# Autodesk Inventor assembly: Walls
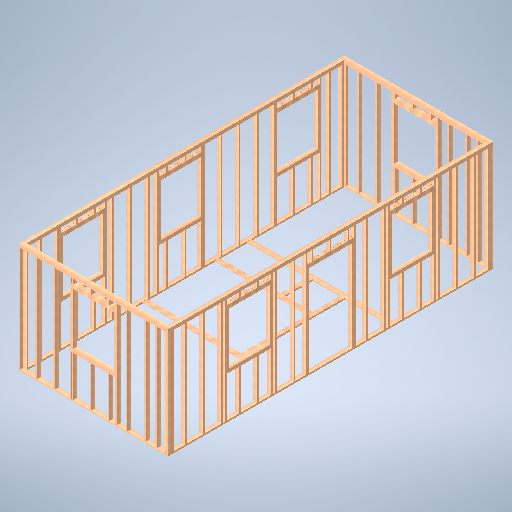
[picture p0: Inventor's stored thumbnail of the model, 512x512]
Saved by Autodesk Inventor 2025.1 (Build 291241020, 241B)
## iProperties
Created: 2024-09-15
Part Number: Walls
Document SubType Name: Assembly
Designer: Tom
Author: Tom
## Documents named in this file (19)
- C:\Users\Tom\Documents\Inventor\Mobility\Additional_Building\Framing_For_First_Floor.iam
- C:\Users\Tom\Documents\Inventor\Mobility\Additional_Building\Plate_With_Length_144_Inches.ipt
- C:\Users\Tom\Documents\Inventor\Mobility\Additional_Building\Plate_With_Length_125_Inches.ipt
- C:\Users\Tom\Documents\Inventor\Mobility\Additional_Building\California_Corner.iam
- C:\Users\Tom\Documents\Inventor\Mobility\Additional_Building\Stud_With_Height_93_Inches.ipt
- C:\Users\Tom\Documents\Inventor\Mobility\Additional_Building\Plate_With_Length_132_Inches.ipt
- C:\Users\Tom\Documents\Inventor\Mobility\Additional_Building\Plate_With_Length_68.5_Inches.ipt
- C:\Users\Tom\Documents\Inventor\Mobility\Additional_Building\Plate_With_Length_86.5625_Inches_And_Image_Of_Bath_Tub.ipt
- C:\Users\Tom\Documents\Inventor\Mobility\Additional_Building\Plate_With_Length_60_Inches.ipt
- C:\Users\Tom\Documents\Inventor\Mobility\Additional_Building\Plate_With_Length_25_Inches.ipt
- C:\Users\Tom\Documents\Inventor\Mobility\Additional_Building\Plate_With_Length_86.5625_Inches.ipt
- C:\Users\Tom\Documents\Inventor\Mobility\Additional_Building\Header_With_Dimensions_3.5_x_3.5_x_41.25_Inches.iam
- C:\Users\Tom\Documents\Inventor\Mobility\Additional_Building\Stud_With_Height_80.5_Inches.ipt
- C:\Users\Tom\Documents\Inventor\Mobility\Additional_Building\Stud_With_Height_9_Inches.ipt
- C:\Users\Tom\Documents\Inventor\Mobility\Additional_Building\Framing_For_First_Floor_Front_Window.iam
- C:\Users\Tom\Documents\Inventor\Mobility\Additional_Building\Framing_For_Side_Window.iam
- C:\Users\Tom\Documents\Inventor\Mobility\Additional_Building\Framing_For_Back_Living_Room_Window.iam
- C:\Users\Tom\Documents\Inventor\Mobility\Additional_Building\Framing_For_Bathroom_Window.iam
- C:\Users\Tom\Documents\Inventor\Mobility\Additional_Building\Framing_For_Back_Bedroom_Window.iam
## Components (74 placed, 18 different names)
1. California_Corner:1 [sub-assembly] — Mate:2, Flush:3, Flush:4
2. California_Corner:2 [sub-assembly] — Mate:13, Flush:13, Flush:14, Flush:19, Flush:20, Flush:31, Mate:34, Flush:64, Flush:70
3. California_Corner:3 [sub-assembly] — Mate:14, Flush:15, Flush:16
4. California_Corner:4 [sub-assembly] — Mate:15, Flush:17, Flush:18, Flush:74, Flush:75
5. Plate_With_Length_125_Inches:5 — Mate:16, Flush:22, Mate:17, Mate:19, Mate:24, Flush:27, Flush:45, Mate:76
6. Plate_With_Length_60_Inches:1 — Mate:19, Mate:27, Mate:31, Flush:44
7. Plate_With_Length_25_Inches:1 — Mate:25, Mate:28, Flush:45
8. Plate_With_Length_25_Inches:2 — Mate:24, Flush:27, Mate:25, Mate:29
9. Plate_With_Length_86.5625_Inches_And_Image_Of_Bath_Tub:1 — Mate:26, Flush:28, Mate:27, Mate:28, Mate:29, Flush:44
10. Plate_With_Length_86.5625_Inches:1 — Mate:30, Mate:31, Flush:29, Mate:73
11. Stud_With_Height_93_Inches:56 — Mate:33, Flush:32, Mate:34, Mate:35, Flush:33, Mate:39
12. Header_With_Dimensions_3.5_x_3.5_x_41.25_Inches:1 [sub-assembly] — Mate:35, Flush:33, Flush:34, Mate:37, Mate:42, Flush:38
13. Stud_With_Height_93_Inches:57 — Mate:36, Flush:35, Mate:37, Mate:41
14. Stud_With_Height_80.5_Inches:1 — Mate:38, Flush:36, Mate:39
15. Stud_With_Height_80.5_Inches:2 — Mate:40, Flush:37, Mate:41
16. Framing_For_First_Floor_Front_Window:1 [sub-assembly] — Mate:62, Flush:63, Flush:64
17. Framing_For_First_Floor_Front_Window:2 [sub-assembly] — Mate:63, Flush:65, Flush:66
18. Stud_With_Height_93_Inches:76 — Mate:67, Flush:73, Flush:74, Flush:79, Flush:83, Flush:85
19. Framing_For_Back_Living_Room_Window:1 [sub-assembly] — Mate:68, Flush:75, Flush:76, Mate:70
20. Stud_With_Height_93_Inches:77 — Mate:69, Flush:77, Mate:70
21. Framing_For_Bathroom_Window:1 [sub-assembly] — Mate:72, Flush:80, Mate:73
22. Framing_For_Back_Bedroom_Window:1 [sub-assembly] — Mate:74, Flush:81, Mate:76
23. Stud_With_Height_93_Inches:84 — Mate:77, Flush:84, Flush:85
24. Plate_With_Length_132_Inches:1 — Mate:8, Flush:9, Flush:10, Mate:10
25. Plate_With_Length_132_Inches:2
26. Plate_With_Length_144_Inches:9 — Mate:11, Mate:12, Flush:12
27. Plate_With_Length_144_Inches:10
28. Stud_With_Height_93_Inches:1 — Mate:4, Flush:6, Flush:19, Flush:39, Flush:43, Flush:68
29. Stud_With_Height_93_Inches:51
30. Stud_With_Height_93_Inches:60 — Flush:62
31. Stud_With_Height_9_Inches:1 — Mate:42, Flush:38, Flush:39
32. Stud_With_Height_9_Inches:2
33. Stud_With_Height_9_Inches:3
34. Stud_With_Height_93_Inches:62 — Mate:61, Flush:61, Flush:62
35. Stud_With_Height_93_Inches:63
36. Stud_With_Height_93_Inches:58 — Mate:44, Flush:42, Flush:43
37. Stud_With_Height_93_Inches:64
38. Stud_With_Height_93_Inches:65 — Mate:64, Flush:67, Flush:68
39. Stud_With_Height_93_Inches:66
40. Stud_With_Height_93_Inches:67
41. Stud_With_Height_93_Inches:49 — Mate:32, Flush:30, Flush:31
42. Framing_For_Side_Window:1 [sub-assembly] — Mate:65, Flush:69, Flush:70
43. Stud_With_Height_93_Inches:71
44. Framing_For_Side_Window:2 [sub-assembly]
45. Stud_With_Height_93_Inches:78 — Mate:71, Flush:78, Flush:79
46. Stud_With_Height_93_Inches:79
47. Stud_With_Height_93_Inches:80
48. Stud_With_Height_93_Inches:81 — Mate:75, Flush:82, Flush:83
49. Stud_With_Height_93_Inches:82
50. Stud_With_Height_93_Inches:83
51. Plate_With_Length_144_Inches:1 — Flush:5, Mate:15, Flush:17, Flush:18, Mate:30, Flush:29, Mate:67, Flush:73, Mate:68, Flush:76, Mate:69, Flush:77, Mate:71, Flush:78, Mate:72, Flush:80
52. Plate_With_Length_144_Inches:2 — Mate:14, Flush:15, Flush:16, Mate:26, Flush:28, Mate:74, Flush:81, Mate:75, Flush:82, Mate:77, Flush:84
53. Plate_With_Length_144_Inches:3 — Mate:1, Flush:1, Flush:2, Mate:4, Flush:6, Mate:13, Flush:13, Flush:14, Mate:16, Flush:22, Mate:33, Flush:32, Flush:34, Mate:38, Flush:36, Mate:61, Flush:61, Mate:62, Flush:63
54. Plate_With_Length_144_Inches:4 — Mate:2, Flush:3, Flush:4, Mate:36, Flush:35, Mate:40, Flush:37, Mate:44, Flush:42, Mate:63, Flush:65, Flush:66, Mate:64, Flush:67
55. Plate_With_Length_125_Inches:1 — Mate:1, Flush:1, Flush:2, Mate:3, Mate:7, Mate:32, Flush:30, Mate:65, Flush:69, Mate:66, Flush:71
56. Plate_With_Length_125_Inches:2 — Mate:17
57. Plate_With_Length_144_Inches:5 — Flush:9
58. Plate_With_Length_144_Inches:6
59. Plate_With_Length_144_Inches:7 — Mate:9, Flush:11
60. Plate_With_Length_144_Inches:8 — Mate:11, Flush:12
61. Plate_With_Length_125_Inches:3 — Flush:7, Mate:8, Flush:10
62. Plate_With_Length_125_Inches:4
63. Plate_With_Length_68.5_Inches:1 — Mate:9, Mate:10, Flush:11
64. Plate_With_Length_68.5_Inches:2 — Mate:12
65. Plate_With_Length_68.5_Inches:3
66. Plate_With_Length_68.5_Inches:4
67. Stud_With_Height_93_Inches:23 — Flush:7, Mate:7, Flush:20, Flush:72
68. Stud_With_Height_93_Inches:68
69. Stud_With_Height_93_Inches:69 — Mate:66, Flush:71, Flush:72
70. Stud_With_Height_93_Inches:70
71. Stud_With_Height_93_Inches:72
72. Stud_With_Height_93_Inches:73
73. Stud_With_Height_93_Inches:74
74. Stud_With_Height_93_Inches:75
## Component patterns: (2 elements), (2 elements, first: Plate_With_Length_132_Inches:1), (2 elements, first: Plate_With_Length_144_Inches:9), (3 elements, first: Stud_With_Height_93_Inches:1), (3 elements, first: Stud_With_Height_9_Inches:1), (2 elements, first: Stud_With_Height_93_Inches:62), (2 elements, first: Stud_With_Height_93_Inches:58), (3 elements, first: Stud_With_Height_93_Inches:65), (2 elements, first: Stud_With_Height_93_Inches:49 + Framing_For_Side_Window:1), (3 elements, first: Stud_With_Height_93_Inches:78), (3 elements, first: Stud_With_Height_93_Inches:81), (4 elements, first: Plate_With_Length_144_Inches:1), (2 elements, first: Plate_With_Length_125_Inches:1), Component Pattern 1:2 (4 elements), Component Pattern 2:2 (2 elements), (2 elements, first: Plate_With_Length_68.5_Inches:1), Component Pattern 10:2 (2 elements), (2 elements, first: Stud_With_Height_93_Inches:23), (2 elements, first: Stud_With_Height_93_Inches:69), Component Pattern 22:2 (2 elements), Component Pattern 23:2 (2 elements)
## Relationships (115: Flush 62, Mate 53)
- Mate:1: Plate_With_Length_144_Inches:3 ↔ Plate_With_Length_125_Inches:1
- Flush:1: Plate_With_Length_144_Inches:3 ↔ Plate_With_Length_125_Inches:1
- Flush:2: Plate_With_Length_144_Inches:3 ↔ Plate_With_Length_125_Inches:1
- Mate:2: California_Corner:1 ↔ Plate_With_Length_144_Inches:4
- Flush:3: California_Corner:1 ↔ Plate_With_Length_144_Inches:4
- Flush:4: California_Corner:1 ↔ Plate_With_Length_144_Inches:4
- Flush:5: Plate_With_Length_144_Inches:1
- Mate:3 (1536.7 mm): Plate_With_Length_125_Inches:1
- Mate:4: Stud_With_Height_93_Inches:1 ↔ Plate_With_Length_144_Inches:3
- Flush:6: Stud_With_Height_93_Inches:1 ↔ Plate_With_Length_144_Inches:3
- Flush:7: Plate_With_Length_125_Inches:3 ↔ Stud_With_Height_93_Inches:23
- Mate:7: Plate_With_Length_125_Inches:1 ↔ Stud_With_Height_93_Inches:23
- Mate:8: Plate_With_Length_132_Inches:1 ↔ Plate_With_Length_125_Inches:3
- Flush:9: Plate_With_Length_132_Inches:1 ↔ Plate_With_Length_144_Inches:5
- Flush:10: Plate_With_Length_132_Inches:1 ↔ Plate_With_Length_125_Inches:3
- Mate:9: Plate_With_Length_144_Inches:7 ↔ Plate_With_Length_68.5_Inches:1
- Mate:10: Plate_With_Length_132_Inches:1 ↔ Plate_With_Length_68.5_Inches:1
- Flush:11: Plate_With_Length_144_Inches:7 ↔ Plate_With_Length_68.5_Inches:1
- Mate:11: Plate_With_Length_144_Inches:9 ↔ Plate_With_Length_144_Inches:8
- Mate:12: Plate_With_Length_144_Inches:9 ↔ Plate_With_Length_68.5_Inches:2
- Flush:12: Plate_With_Length_144_Inches:9 ↔ Plate_With_Length_144_Inches:8
- Mate:13: California_Corner:2 ↔ Plate_With_Length_144_Inches:3
- Flush:13: California_Corner:2 ↔ Plate_With_Length_144_Inches:3
- Flush:14: California_Corner:2 ↔ Plate_With_Length_144_Inches:3
- Mate:14: California_Corner:3 ↔ Plate_With_Length_144_Inches:2
- Flush:15: California_Corner:3 ↔ Plate_With_Length_144_Inches:2
- Flush:16: California_Corner:3 ↔ Plate_With_Length_144_Inches:2
- Mate:15: California_Corner:4 ↔ Plate_With_Length_144_Inches:1
- Flush:17: California_Corner:4 ↔ Plate_With_Length_144_Inches:1
- Flush:18: California_Corner:4 ↔ Plate_With_Length_144_Inches:1
- Flush:19 (387.35 mm): California_Corner:2 ↔ Stud_With_Height_93_Inches:1
- Flush:20 (501.65 mm): California_Corner:2 ↔ Stud_With_Height_93_Inches:23
- Mate:16: Plate_With_Length_125_Inches:5 ↔ Plate_With_Length_144_Inches:3
- Flush:22: Plate_With_Length_125_Inches:5 ↔ Plate_With_Length_144_Inches:3
- Mate:17 (2092.325 mm): Plate_With_Length_125_Inches:5 ↔ Plate_With_Length_125_Inches:2
- Mate:19 (723.9 mm): Plate_With_Length_125_Inches:5 ↔ Plate_With_Length_60_Inches:1
- Mate:24: Plate_With_Length_125_Inches:5 ↔ Plate_With_Length_25_Inches:2
- Flush:27: Plate_With_Length_125_Inches:5 ↔ Plate_With_Length_25_Inches:2
- Mate:25 (635 mm): Plate_With_Length_25_Inches:1 ↔ Plate_With_Length_25_Inches:2
- Mate:26: Plate_With_Length_86.5625_Inches_And_Image_Of_Bath_Tub:1 ↔ Plate_With_Length_144_Inches:2
- Flush:28: Plate_With_Length_86.5625_Inches_And_Image_Of_Bath_Tub:1 ↔ Plate_With_Length_144_Inches:2
- Mate:27: Plate_With_Length_60_Inches:1 ↔ Plate_With_Length_86.5625_Inches_And_Image_Of_Bath_Tub:1
- Mate:28: Plate_With_Length_25_Inches:1 ↔ Plate_With_Length_86.5625_Inches_And_Image_Of_Bath_Tub:1
- Mate:29: Plate_With_Length_25_Inches:2 ↔ Plate_With_Length_86.5625_Inches_And_Image_Of_Bath_Tub:1
- Mate:30: Plate_With_Length_86.5625_Inches:1 ↔ Plate_With_Length_144_Inches:1
- Mate:31: Plate_With_Length_60_Inches:1 ↔ Plate_With_Length_86.5625_Inches:1
- Flush:29: Plate_With_Length_86.5625_Inches:1 ↔ Plate_With_Length_144_Inches:1
- Mate:32: Stud_With_Height_93_Inches:49 ↔ Plate_With_Length_125_Inches:1
- Flush:30: Stud_With_Height_93_Inches:49 ↔ Plate_With_Length_125_Inches:1
- Flush:31 (250.825 mm): California_Corner:2 ↔ Stud_With_Height_93_Inches:49
- Mate:33: Stud_With_Height_93_Inches:56 ↔ Plate_With_Length_144_Inches:3
- Flush:32: Stud_With_Height_93_Inches:56 ↔ Plate_With_Length_144_Inches:3
- Mate:34 (-3133.725 mm): California_Corner:2 ↔ Stud_With_Height_93_Inches:56
- Mate:35: Stud_With_Height_93_Inches:56 ↔ Header_With_Dimensions_3.5_x_3.5_x_41.25_Inches:1
- Flush:33: Stud_With_Height_93_Inches:56 ↔ Header_With_Dimensions_3.5_x_3.5_x_41.25_Inches:1
- Flush:34 (2082.8 mm): Header_With_Dimensions_3.5_x_3.5_x_41.25_Inches:1 ↔ Plate_With_Length_144_Inches:3
- Mate:36: Stud_With_Height_93_Inches:57 ↔ Plate_With_Length_144_Inches:4
- Flush:35: Stud_With_Height_93_Inches:57 ↔ Plate_With_Length_144_Inches:4
- Mate:37: Header_With_Dimensions_3.5_x_3.5_x_41.25_Inches:1 ↔ Stud_With_Height_93_Inches:57
- Mate:38: Stud_With_Height_80.5_Inches:1 ↔ Plate_With_Length_144_Inches:3
- Flush:36: Stud_With_Height_80.5_Inches:1 ↔ Plate_With_Length_144_Inches:3
- Mate:39: Stud_With_Height_93_Inches:56 ↔ Stud_With_Height_80.5_Inches:1
- Mate:40: Stud_With_Height_80.5_Inches:2 ↔ Plate_With_Length_144_Inches:4
- Flush:37: Stud_With_Height_80.5_Inches:2 ↔ Plate_With_Length_144_Inches:4
- Mate:41: Stud_With_Height_93_Inches:57 ↔ Stud_With_Height_80.5_Inches:2
- Mate:42: Header_With_Dimensions_3.5_x_3.5_x_41.25_Inches:1 ↔ Stud_With_Height_9_Inches:1
- Flush:38: Header_With_Dimensions_3.5_x_3.5_x_41.25_Inches:1 ↔ Stud_With_Height_9_Inches:1
- Flush:39 (2844.8 mm): Stud_With_Height_93_Inches:1 ↔ Stud_With_Height_9_Inches:1
- Mate:44: Stud_With_Height_93_Inches:58 ↔ Plate_With_Length_144_Inches:4
- Flush:42: Stud_With_Height_93_Inches:58 ↔ Plate_With_Length_144_Inches:4
- Flush:43 (4064 mm): Stud_With_Height_93_Inches:1 ↔ Stud_With_Height_93_Inches:58
- Flush:44: Plate_With_Length_60_Inches:1 ↔ Plate_With_Length_86.5625_Inches_And_Image_Of_Bath_Tub:1
- Flush:45: Plate_With_Length_125_Inches:5 ↔ Plate_With_Length_25_Inches:1
- Mate:61: Stud_With_Height_93_Inches:62 ↔ Plate_With_Length_144_Inches:3
- Flush:61: Stud_With_Height_93_Inches:62 ↔ Plate_With_Length_144_Inches:3
- Flush:62 (1219.2 mm): Stud_With_Height_93_Inches:60 ↔ Stud_With_Height_93_Inches:62
- Mate:62: Framing_For_First_Floor_Front_Window:1 ↔ Plate_With_Length_144_Inches:3
- Flush:63: Framing_For_First_Floor_Front_Window:1 ↔ Plate_With_Length_144_Inches:3
- Flush:64 (1295.4 mm): California_Corner:2 ↔ Framing_For_First_Floor_Front_Window:1
- Mate:63: Framing_For_First_Floor_Front_Window:2 ↔ Plate_With_Length_144_Inches:4
- Flush:65: Framing_For_First_Floor_Front_Window:2 ↔ Plate_With_Length_144_Inches:4
- Flush:66 (-1295.4 mm): Framing_For_First_Floor_Front_Window:2 ↔ Plate_With_Length_144_Inches:4
- Mate:64: Stud_With_Height_93_Inches:65 ↔ Plate_With_Length_144_Inches:4
- Flush:67: Stud_With_Height_93_Inches:65 ↔ Plate_With_Length_144_Inches:4
- Flush:68 (5689.6 mm): Stud_With_Height_93_Inches:1 ↔ Stud_With_Height_93_Inches:65
- Mate:65: Framing_For_Side_Window:1 ↔ Plate_With_Length_125_Inches:1
- Flush:69: Framing_For_Side_Window:1 ↔ Plate_With_Length_125_Inches:1
- Flush:70 (1143 mm): California_Corner:2 ↔ Framing_For_Side_Window:1
- Mate:66: Plate_With_Length_125_Inches:1 ↔ Stud_With_Height_93_Inches:69
- Flush:71: Plate_With_Length_125_Inches:1 ↔ Stud_With_Height_93_Inches:69
- Flush:72 (2032 mm): Stud_With_Height_93_Inches:23 ↔ Stud_With_Height_93_Inches:69
- Mate:67: Stud_With_Height_93_Inches:76 ↔ Plate_With_Length_144_Inches:1
- Flush:73: Stud_With_Height_93_Inches:76 ↔ Plate_With_Length_144_Inches:1
- Flush:74 (387.35 mm): California_Corner:4 ↔ Stud_With_Height_93_Inches:76
- Mate:68: Framing_For_Back_Living_Room_Window:1 ↔ Plate_With_Length_144_Inches:1
- Flush:75 (820.7375 mm): California_Corner:4 ↔ Framing_For_Back_Living_Room_Window:1
- Flush:76: Framing_For_Back_Living_Room_Window:1 ↔ Plate_With_Length_144_Inches:1
- Mate:69: Stud_With_Height_93_Inches:77 ↔ Plate_With_Length_144_Inches:1
- Flush:77: Stud_With_Height_93_Inches:77 ↔ Plate_With_Length_144_Inches:1
- Mate:70: Framing_For_Back_Living_Room_Window:1 ↔ Stud_With_Height_93_Inches:77
- Mate:71: Stud_With_Height_93_Inches:78 ↔ Plate_With_Length_144_Inches:1
- Flush:78: Stud_With_Height_93_Inches:78 ↔ Plate_With_Length_144_Inches:1
- Flush:79 (1625.6 mm): Stud_With_Height_93_Inches:76 ↔ Stud_With_Height_93_Inches:78
- Mate:72: Framing_For_Bathroom_Window:1 ↔ Plate_With_Length_144_Inches:1
- Flush:80: Framing_For_Bathroom_Window:1 ↔ Plate_With_Length_144_Inches:1
- Mate:73 (228.6 mm): Plate_With_Length_86.5625_Inches:1 ↔ Framing_For_Bathroom_Window:1
- Mate:74: Framing_For_Back_Bedroom_Window:1 ↔ Plate_With_Length_144_Inches:2
- Flush:81: Framing_For_Back_Bedroom_Window:1 ↔ Plate_With_Length_144_Inches:2
- Mate:75: Stud_With_Height_93_Inches:81 ↔ Plate_With_Length_144_Inches:2
- Flush:82: Stud_With_Height_93_Inches:81 ↔ Plate_With_Length_144_Inches:2
- Flush:83 (4064 mm): Stud_With_Height_93_Inches:76 ↔ Stud_With_Height_93_Inches:81
- Mate:76 (512.7625 mm): Plate_With_Length_125_Inches:5 ↔ Framing_For_Back_Bedroom_Window:1
- Mate:77: Stud_With_Height_93_Inches:84 ↔ Plate_With_Length_144_Inches:2
- Flush:84: Stud_With_Height_93_Inches:84 ↔ Plate_With_Length_144_Inches:2
- Flush:85 (6502.4 mm): Stud_With_Height_93_Inches:76 ↔ Stud_With_Height_93_Inches:84
